# Autodesk Inventor assembly: Assembly1
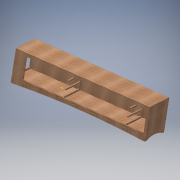
[picture p0: Inventor's stored thumbnail of the model, 180x180]
Saved by Autodesk Inventor 2016 (Build 200138000, 138)
## iProperties
Created: 2017-02-03
Part Number: Assembly1
Document SubType Name: Assembly
Designer: jwillauer
Author: jwillauer
## Documents named in this file (8)
- D:\New folder\87\Assembly1.iam
- D:\New folder\87\back.ipt
- D:\New folder\87\front.ipt
- D:\New folder\87\right side.ipt
- D:\New folder\87\bottom.ipt
- D:\New folder\87\snowboard rack.ipt
- D:\New folder\87\top.ipt
- D:\New folder\87\left side.ipt
## Components (8 placed, 7 different names)
1. back:1 — Flush:3, Flush:4, Flush:5, Flush:7, Mate:1, Mate:2, Mate:7, Flush:9
2. front:1 — Flush:2, Flush:8, Flush:10, Mate:8, Flush:11, Flush:12
3. right side:1 — Flush:2, Flush:3, Flush:4, Flush:5, Flush:6, Mate:5, Flush:8
4. bottom:1 — Flush:6, Flush:7, Mate:3, Mate:4
5. snowboard rack:1 — Mate:2, Mate:3, Mate:6
6. snowboard rack:2 — Mate:1, Mate:4, Mate:5, Mate:6
7. top:1 — Mate:7, Flush:9, Flush:10
8. left side:1 — Mate:8, Flush:11, Flush:12
## Relationships (19: Flush 11, Mate 8)
- Flush:2: front:1 ↔ right side:1
- Flush:3: back:1 ↔ right side:1
- Flush:4: back:1 ↔ right side:1
- Flush:5: back:1 ↔ right side:1
- Flush:6: right side:1 ↔ bottom:1
- Flush:7: back:1 ↔ bottom:1
- Mate:1: back:1 ↔ snowboard rack:2
- Mate:2: back:1 ↔ snowboard rack:1
- Mate:3: bottom:1 ↔ snowboard rack:1
- Mate:4: bottom:1 ↔ snowboard rack:2
- Mate:5 (304.8 mm): right side:1 ↔ snowboard rack:2
- Mate:6 (914.4 mm): snowboard rack:1 ↔ snowboard rack:2
- Flush:8: front:1 ↔ right side:1
- Mate:7: back:1 ↔ top:1
- Flush:9: back:1 ↔ top:1
- Flush:10: front:1 ↔ top:1
- Mate:8: front:1 ↔ left side:1
- Flush:11: front:1 ↔ left side:1
- Flush:12: front:1 ↔ left side:1
